# Autodesk Inventor assembly: C-Beam Gantry Plate Assy
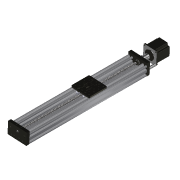
[picture p0: Inventor's stored thumbnail of the model, 180x180]
Saved by Autodesk Inventor 2019 (Build 230136000, 136)
## iProperties
Created: 2020-11-22
Part Number: C-Beam Gantry Plate Assy
Document SubType Name: Assembly
Designer: asus
Author: asus
## Documents named in this file (22)
- F:\R o n i\GrabCAD\Linear actuator [Open Build]\Autodesk Inventor File\Linear actuator [Open Build].iam
- F:\R o n i\GrabCAD\Linear actuator [Open Build]\Autodesk Inventor File\Aluminium Spacer 3mm.ipt
- F:\R o n i\GrabCAD\Linear actuator [Open Build]\Autodesk Inventor File\Aluminium Spacer 6mm.ipt
- F:\R o n i\GrabCAD\Linear actuator [Open Build]\Autodesk Inventor File\Ball Bearing 5 x 10 x 4.2.ipt
- F:\R o n i\GrabCAD\Linear actuator [Open Build]\Autodesk Inventor File\C-Beam Gantry Plate.ipt
- F:\R o n i\GrabCAD\Linear actuator [Open Build]\Autodesk Inventor File\Low Profile Screw M5 [20mm].ipt
- F:\R o n i\GrabCAD\Linear actuator [Open Build]\Autodesk Inventor File\Low Profile Screw M5 [25mm].ipt
- F:\R o n i\GrabCAD\Linear actuator [Open Build]\Autodesk Inventor File\Mini Eccentric Spacer 6mm.ipt
- F:\R o n i\GrabCAD\Linear actuator [Open Build]\Autodesk Inventor File\Nylon Insert Lock Nut M5.ipt
- F:\R o n i\GrabCAD\Linear actuator [Open Build]\Autodesk Inventor File\Precision Shim 8 x 5 x 1.ipt
- F:\R o n i\GrabCAD\Linear actuator [Open Build]\Autodesk Inventor File\Xtreme Mini V Wheel.ipt
- F:\R o n i\GrabCAD\Linear actuator [Open Build]\Autodesk Inventor File\Anti-Backlash Nut Block.ipt
- C:\Users\Roni Mahendra\Documents\Inventor\Content Center Files\R2019\en-US\AS 1421(2)\AS 1421 - M5 x 12 Cup Point.ipt
- F:\R o n i\GrabCAD\Linear actuator [Open Build]\Autodesk Inventor File\C-Beam End Mount.ipt
- F:\R o n i\GrabCAD\Linear actuator [Open Build]\Autodesk Inventor File\C-Beam 4080 500mm.ipt
- F:\R o n i\GrabCAD\Linear actuator [Open Build]\Autodesk Inventor File\Nema 23.ipt
- C:\Users\Roni Mahendra\Documents\Inventor\Content Center Files\R2019\en-US\AS 1420\AS 1420 - 1973 - M3 x 12.ipt
- F:\R o n i\GrabCAD\Linear actuator [Open Build]\Autodesk Inventor File\Ball Screw [540mm].ipt
- F:\R o n i\GrabCAD\Linear actuator [Open Build]\Autodesk Inventor File\Ball Bearing 8 x 16 x 5.ipt
- F:\R o n i\GrabCAD\Linear actuator [Open Build]\Autodesk Inventor File\Lock Collar 8mm.ipt
- F:\R o n i\GrabCAD\Linear actuator [Open Build]\Autodesk Inventor File\Shim Washer 8mm.ipt
- C:\Users\Roni Mahendra\Documents\Inventor\Content Center Files\R2019\en-US\AS 1421(2)\AS 1421 - M4 x 5 Cup Point.ipt
## Components (64 placed, 21 different names)
1. Aluminium Spacer 3mm:1 — Insert:35, Insert:37
2. Aluminium Spacer 6mm:1 — Insert:3, Insert:4
3. Ball Bearing 5 x 10 x 4.2:1 — Insert:5, Insert:6
4. C-Beam Gantry Plate:1 — Insert:1, Insert:2, Insert:3, Insert:10, Insert:17, Insert:18, Insert:19, Insert:26, Insert:33, Insert:34, Insert:35, Insert:36, Angle:1
5. Low Profile Screw M5 [20mm]:1 — Insert:34, Mate:1
6. Low Profile Screw M5 [25mm]:1 — Insert:1
7. Mini Eccentric Spacer 6mm:1 — Insert:10, Insert:11
8. Nylon Insert Lock Nut M5:1 — Insert:9
9. Precision Shim 8 x 5 x 1:1 — Insert:4, Insert:5
10. Xtreme Mini V Wheel:1 — Insert:6, Insert:7, Insert:8
11. Aluminium Spacer 3mm:2 — Insert:36
12. Aluminium Spacer 6mm:2 — Insert:19, Insert:20
13. Anti-Backlash Nut Block:1 — Insert:37, Mate:1, Insert:38, Insert:39, Insert:40, Mate:6
14. Ball Bearing 5 x 10 x 4.2:2 — Insert:8, Insert:9
15. Low Profile Screw M5 [20mm]:2 — Insert:33
16. Low Profile Screw M5 [25mm]:2 — Insert:2
17. Mini Eccentric Spacer 6mm:2 — Insert:26, Insert:27
18. Nylon Insert Lock Nut M5:2 — Insert:39
19. Precision Shim 8 x 5 x 1:2 — Insert:7
20. Xtreme Mini V Wheel:2 — Insert:29, Insert:30, Insert:31
21. Ball Bearing 5 x 10 x 4.2:3 — Insert:12, Insert:13
22. Ball Bearing 5 x 10 x 4.2:4 — Insert:15, Insert:16
23. Ball Bearing 5 x 10 x 4.2:5 — Insert:31, Insert:32
24. Ball Bearing 5 x 10 x 4.2:6 — Insert:28, Insert:29
25. Ball Bearing 5 x 10 x 4.2:7 — Insert:24, Insert:25
26. Ball Bearing 5 x 10 x 4.2:8 — Insert:21, Insert:22
27. Low Profile Screw M5 [25mm]:3 — Insert:18
28. Low Profile Screw M5 [25mm]:4 — Insert:17
29. Nylon Insert Lock Nut M5:3 — Insert:38
30. Nylon Insert Lock Nut M5:4 — Insert:16
31. Nylon Insert Lock Nut M5:5 — Insert:32
32. Nylon Insert Lock Nut M5:6 — Insert:25
33. Precision Shim 8 x 5 x 1:3 — Insert:20, Insert:21
34. Precision Shim 8 x 5 x 1:4 — Insert:14
35. Precision Shim 8 x 5 x 1:5 — Insert:11, Insert:12
36. Precision Shim 8 x 5 x 1:6 — Insert:23
37. Precision Shim 8 x 5 x 1:7 — Insert:30
38. Precision Shim 8 x 5 x 1:8 — Insert:27, Insert:28
39. Xtreme Mini V Wheel:3 — Insert:22, Insert:23, Insert:24
40. Xtreme Mini V Wheel:4 — Insert:13, Insert:14, Insert:15
41. AS 1421 Cup Point - Metric M5 x 12 Cup Point:1 — Insert:40
42. C-Beam End Mount:1 — Insert:42, Insert:43, Insert:48, Insert:49, Insert:50, Insert:51, Insert:60, Insert:61
43. C-Beam End Mount:2 — Insert:41, Mate:2, Insert:44, Insert:45, Insert:46, Insert:47, Insert:52, Mate:3, Insert:54
44. C-Beam 4080 500mm:1 — Insert:41, Insert:42, Insert:43, Mate:2, Angle:1
45. Low Profile Screw M5 [20mm]:3 — Insert:46
46. Low Profile Screw M5 [20mm]:4 — Insert:45
47. Low Profile Screw M5 [20mm]:5 — Insert:44
48. Low Profile Screw M5 [20mm]:6 — Insert:47
49. Low Profile Screw M5 [20mm]:7 — Insert:49
50. Low Profile Screw M5 [20mm]:8 — Insert:50
51. Low Profile Screw M5 [20mm]:9 — Insert:48
52. Low Profile Screw M5 [20mm]:10 — Insert:51
53. Nema 23:1 — Insert:52, Mate:3, Insert:53, Mate:4, Mate:5
54. AS 1420 - Metric M3 x 12:1 — Insert:53
55. AS 1420 - Metric M3 x 12:2 — Mate:4, Mate:5
56. Ball Screw [540mm]:1 — Insert:61, Mate:6
57. Ball Bearing 8 x 16 x 5:1 — Insert:54, Insert:57
58. Ball Bearing 8 x 16 x 5:2 — Insert:56, Insert:60
59. Lock Collar 8mm:1 — Insert:58, Mate:8, Tangent:1
60. Lock Collar 8mm:2 — Insert:59, Mate:7, Tangent:2
61. Shim Washer 8mm:1 — Insert:57, Insert:58
62. Shim Washer 8mm:2 — Insert:56, Insert:59
63. AS 1421 Cup Point - Metric M4 x 5 Cup Point:2 — Mate:7, Tangent:2
64. AS 1421 Cup Point - Metric M4 x 5 Cup Point:1 — Mate:8, Tangent:1
## Relationships (71: Insert 60, Mate 8, Tangent 2, Angle 1)
- Insert:1: C-Beam Gantry Plate:1 ↔ Low Profile Screw M5 [25mm]:1
- Insert:2: C-Beam Gantry Plate:1 ↔ Low Profile Screw M5 [25mm]:2
- Insert:3: Aluminium Spacer 6mm:1 ↔ C-Beam Gantry Plate:1
- Insert:4: Aluminium Spacer 6mm:1 ↔ Precision Shim 8 x 5 x 1:1
- Insert:5: Ball Bearing 5 x 10 x 4.2:1 ↔ Precision Shim 8 x 5 x 1:1
- Insert:6: Ball Bearing 5 x 10 x 4.2:1 ↔ Xtreme Mini V Wheel:1
- Insert:7: Xtreme Mini V Wheel:1 ↔ Precision Shim 8 x 5 x 1:2
- Insert:8: Xtreme Mini V Wheel:1 ↔ Ball Bearing 5 x 10 x 4.2:2
- Insert:9: Nylon Insert Lock Nut M5:1 ↔ Ball Bearing 5 x 10 x 4.2:2
- Insert:10: C-Beam Gantry Plate:1 ↔ Mini Eccentric Spacer 6mm:1
- Insert:11: Mini Eccentric Spacer 6mm:1 ↔ Precision Shim 8 x 5 x 1:5
- Insert:12: Ball Bearing 5 x 10 x 4.2:3 ↔ Precision Shim 8 x 5 x 1:5
- Insert:13: Ball Bearing 5 x 10 x 4.2:3 ↔ Xtreme Mini V Wheel:4
- Insert:14: Precision Shim 8 x 5 x 1:4 ↔ Xtreme Mini V Wheel:4
- Insert:15: Ball Bearing 5 x 10 x 4.2:4 ↔ Xtreme Mini V Wheel:4
- Insert:16: Ball Bearing 5 x 10 x 4.2:4 ↔ Nylon Insert Lock Nut M5:4
- Insert:17: C-Beam Gantry Plate:1 ↔ Low Profile Screw M5 [25mm]:4
- Insert:18: C-Beam Gantry Plate:1 ↔ Low Profile Screw M5 [25mm]:3
- Insert:19: C-Beam Gantry Plate:1 ↔ Aluminium Spacer 6mm:2
- Insert:20: Aluminium Spacer 6mm:2 ↔ Precision Shim 8 x 5 x 1:3
- Insert:21: Ball Bearing 5 x 10 x 4.2:8 ↔ Precision Shim 8 x 5 x 1:3
- Insert:22: Ball Bearing 5 x 10 x 4.2:8 ↔ Xtreme Mini V Wheel:3
- Insert:23: Precision Shim 8 x 5 x 1:6 ↔ Xtreme Mini V Wheel:3
- Insert:24: Ball Bearing 5 x 10 x 4.2:7 ↔ Xtreme Mini V Wheel:3
- Insert:25: Ball Bearing 5 x 10 x 4.2:7 ↔ Nylon Insert Lock Nut M5:6
- Insert:26: C-Beam Gantry Plate:1 ↔ Mini Eccentric Spacer 6mm:2
- Insert:27: Mini Eccentric Spacer 6mm:2 ↔ Precision Shim 8 x 5 x 1:8
- Insert:28: Ball Bearing 5 x 10 x 4.2:6 ↔ Precision Shim 8 x 5 x 1:8
- Insert:29: Xtreme Mini V Wheel:2 ↔ Ball Bearing 5 x 10 x 4.2:6
- Insert:30: Xtreme Mini V Wheel:2 ↔ Precision Shim 8 x 5 x 1:7
- Insert:31: Xtreme Mini V Wheel:2 ↔ Ball Bearing 5 x 10 x 4.2:5
- Insert:32: Ball Bearing 5 x 10 x 4.2:5 ↔ Nylon Insert Lock Nut M5:5
- Insert:33: C-Beam Gantry Plate:1 ↔ Low Profile Screw M5 [20mm]:2
- Insert:34: C-Beam Gantry Plate:1 ↔ Low Profile Screw M5 [20mm]:1
- Insert:35: Aluminium Spacer 3mm:1 ↔ C-Beam Gantry Plate:1
- Insert:36: C-Beam Gantry Plate:1 ↔ Aluminium Spacer 3mm:2
- Insert:37 (0.3 mm): Aluminium Spacer 3mm:1 ↔ Anti-Backlash Nut Block:1
- Mate:1: Low Profile Screw M5 [20mm]:1 ↔ Anti-Backlash Nut Block:1
- Insert:38: Anti-Backlash Nut Block:1 ↔ Nylon Insert Lock Nut M5:3
- Insert:39: Anti-Backlash Nut Block:1 ↔ Nylon Insert Lock Nut M5:2
- Insert:40: Anti-Backlash Nut Block:1 ↔ AS 1421 Cup Point - Metric M5 x 12 Cup Point:1
- Insert:41: C-Beam End Mount:2 ↔ C-Beam 4080 500mm:1
- Insert:42: C-Beam End Mount:1 ↔ C-Beam 4080 500mm:1
- Insert:43: C-Beam End Mount:1 ↔ C-Beam 4080 500mm:1
- Mate:2: C-Beam End Mount:2 ↔ C-Beam 4080 500mm:1
- Insert:44: C-Beam End Mount:2 ↔ Low Profile Screw M5 [20mm]:5
- Insert:45: C-Beam End Mount:2 ↔ Low Profile Screw M5 [20mm]:4
- Insert:46: C-Beam End Mount:2 ↔ Low Profile Screw M5 [20mm]:3
- Insert:47: C-Beam End Mount:2 ↔ Low Profile Screw M5 [20mm]:6
- Insert:48: C-Beam End Mount:1 ↔ Low Profile Screw M5 [20mm]:9
- Insert:49: C-Beam End Mount:1 ↔ Low Profile Screw M5 [20mm]:7
- Insert:50: C-Beam End Mount:1 ↔ Low Profile Screw M5 [20mm]:8
- Insert:51: C-Beam End Mount:1 ↔ Low Profile Screw M5 [20mm]:10
- Insert:52: C-Beam End Mount:2 ↔ Nema 23:1
- Mate:3: C-Beam End Mount:2 ↔ Nema 23:1
- Insert:53: Nema 23:1 ↔ AS 1420 - Metric M3 x 12:1
- Mate:4: Nema 23:1 ↔ AS 1420 - Metric M3 x 12:2
- Mate:5: Nema 23:1 ↔ AS 1420 - Metric M3 x 12:2
- Insert:54: C-Beam End Mount:2 ↔ Ball Bearing 8 x 16 x 5:1
- Insert:56: Ball Bearing 8 x 16 x 5:2 ↔ Shim Washer 8mm:2
- Insert:57: Ball Bearing 8 x 16 x 5:1 ↔ Shim Washer 8mm:1
- Insert:58: Lock Collar 8mm:1 ↔ Shim Washer 8mm:1
- Insert:59: Lock Collar 8mm:2 ↔ Shim Washer 8mm:2
- Insert:60: C-Beam End Mount:1 ↔ Ball Bearing 8 x 16 x 5:2
- Insert:61: C-Beam End Mount:1 ↔ Ball Screw [540mm]:1
- Mate:6: Anti-Backlash Nut Block:1 ↔ Ball Screw [540mm]:1
- Angle:1 (0 deg): C-Beam Gantry Plate:1 ↔ C-Beam 4080 500mm:1
- Mate:7: Lock Collar 8mm:2 ↔ AS 1421 Cup Point - Metric M4 x 5 Cup Point:2
- Mate:8: Lock Collar 8mm:1 ↔ AS 1421 Cup Point - Metric M4 x 5 Cup Point:1
- Tangent:1: Lock Collar 8mm:1 ↔ AS 1421 Cup Point - Metric M4 x 5 Cup Point:1
- Tangent:2: Lock Collar 8mm:2 ↔ AS 1421 Cup Point - Metric M4 x 5 Cup Point:2
